# Autodesk Inventor assembly: SleepingWingLinkage
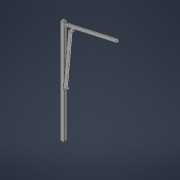
[picture p0: Inventor's stored thumbnail of the model, 180x180]
Saved by Autodesk Inventor 2021 (Build 250183000, 183)
## iProperties
Created: 2021-01-30
Part Number: SleepingWingLinkage
Document SubType Name: Assembly
Designer: argon
Author: argon
## Documents named in this file (5)
- C:\Users\argon\OneDrive\Documents\GrabCAD\EngOne Maroons\Prototype Mechanisms\Seat Sleeping Wings\SleepingWingLinkage.iam
- C:\Users\argon\OneDrive\Documents\GrabCAD\EngOne Maroons\Prototype Mechanisms\Seat Sleeping Wings\LinearRail.ipt
- C:\Users\argon\OneDrive\Documents\GrabCAD\EngOne Maroons\Prototype Mechanisms\Seat Sleeping Wings\Wing.ipt
- C:\Users\argon\OneDrive\Documents\GrabCAD\EngOne Maroons\Prototype Mechanisms\Seat Sleeping Wings\LinearSlider.ipt
- C:\Users\argon\OneDrive\Documents\GrabCAD\EngOne Maroons\Prototype Mechanisms\Seat Sleeping Wings\LongLink.ipt
## Components (5 placed, 4 different names)
1. LinearRail:1 — Mate:1, Mate:2, Mate:5, Mate:6
2. Wing:1 — Mate:7, Mate:8, Mate:9
3. LinearSlider:1 — Mate:1, Mate:2, Mate:3, Mate:4
4. LongLink:1 — Mate:3, Mate:4, Mate:9
5. LinearSlider:2 — Mate:5, Mate:6, Mate:7, Mate:8
## Relationships (9: Mate 9)
- Mate:1: LinearRail:1 ↔ LinearSlider:1
- Mate:2: LinearRail:1 ↔ LinearSlider:1
- Mate:3: LinearSlider:1 ↔ LongLink:1
- Mate:4: LinearSlider:1 ↔ LongLink:1
- Mate:5: LinearRail:1 ↔ LinearSlider:2
- Mate:6: LinearRail:1 ↔ LinearSlider:2
- Mate:7: Wing:1 ↔ LinearSlider:2
- Mate:8: Wing:1 ↔ LinearSlider:2
- Mate:9: Wing:1 ↔ LongLink:1
